# Autodesk Inventor assembly: Case
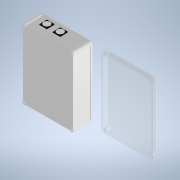
[picture p0: Inventor's stored thumbnail of the model, 180x180]
Saved by Autodesk Inventor 2020 (Build 240168000, 168)
## iProperties
Created: 2019-12-11
Part Number: Case
Document SubType Name: Assembly
Designer: nicoc
Author: nicoc
## Documents named in this file (12)
- D:\Repos\P5-AIonFPGA\cad\Case\Case.iam
- D:\Repos\P5-AIonFPGA\cad\Case\Ultra96\PWB_USDEV1-1_FINAL.iam
- D:\Repos\P5-AIonFPGA\cad\Case\Terminalblock\Terminalblock.iam
- D:\Repos\P5-AIonFPGA\cad\Case\SlottedWiring\SlottexWiring200mm.ipt
- D:\Repos\P5-AIonFPGA\cad\Case\SlottedWiring\SlottexWiring110mm.ipt
- D:\Repos\P5-AIonFPGA\cad\Case\Ventilator\Filter.ipt
- D:\Repos\P5-AIonFPGA\cad\Case\Fibox_PC_3828 _3_T_Bottom.ipt
- D:\Repos\P5-AIonFPGA\cad\Case\Fibox_PC_3828 _3_T_Top.ipt
- D:\Repos\P5-AIonFPGA\cad\Case\Ventilator\Fan_40x40x20.iam
- D:\Repos\P5-AIonFPGA\cad\Case\Ventilator\Filter40x40x20.ipt
- D:\Repos\P5-AIonFPGA\cad\Case\Ventilator\Fan_60x60x25.ipt
- D:\Repos\P5-AIonFPGA\cad\Case\Ultra96\USBCable.ipt
## Components (15 placed, 11 different names)
1. PWB_USDEV1-1_FINAL:1 [sub-assembly] — Mate:4, Mate:5, Mate:8, Mate:23, Flush:20, Flush:21
2. Terminalblock:1 [sub-assembly] — Mate:6, Mate:7
3. SlottexWiring200mm:1 — Mate:2, Flush:2, Flush:3, Flush:4
4. SlottexWiring200mm:2 — Mate:1, Flush:1, Flush:4, Mate:7, Mate:8
5. SlottexWiring110mm:1 — Mate:1, Flush:1, Mate:2, Flush:2, Flush:3, Mate:3, Mate:5
6. Filter:1 — Mate:15
7. Filter:2 — Mate:14, Mate:22, Flush:18, Flush:19
8. Fibox_PC_3828 _3_T_Bottom:1 — Mate:3, Mate:4, Mate:6, Mate:14, Mate:15, Mate:16, Mate:20, Mate:21
9. Fibox_PC_3828 _3_T_Top:1 — Mate:21
10. Fan_40x40x20:1 [sub-assembly] — Mate:17, Flush:11, Flush:12
11. Filter40x40x20:1 — Mate:16, Mate:17, Flush:11, Flush:12, Flush:17
12. Fan_40x40x20:3 [sub-assembly]
13. Filter40x40x20:3 — Mate:20, Flush:17
14. Fan_60x60x25:1 — Mate:22, Flush:18, Flush:19
15. USBCable:1 — Mate:23, Flush:20, Flush:21
## Relationships (30: Mate 17, Flush 13)
- Mate:1: SlottexWiring200mm:2 ↔ SlottexWiring110mm:1
- Flush:1: SlottexWiring200mm:2 ↔ SlottexWiring110mm:1
- Mate:2: SlottexWiring200mm:1 ↔ SlottexWiring110mm:1
- Flush:2: SlottexWiring200mm:1 ↔ SlottexWiring110mm:1
- Flush:3: SlottexWiring200mm:1 ↔ SlottexWiring110mm:1
- Flush:4: SlottexWiring200mm:1 ↔ SlottexWiring200mm:2
- Mate:3: SlottexWiring110mm:1 ↔ Fibox_PC_3828 _3_T_Bottom:1
- Mate:4: PWB_USDEV1-1_FINAL:1 ↔ Fibox_PC_3828 _3_T_Bottom:1
- Mate:5 (40 mm): PWB_USDEV1-1_FINAL:1 ↔ SlottexWiring110mm:1
- Mate:6: Terminalblock:1 ↔ Fibox_PC_3828 _3_T_Bottom:1
- Mate:7 (10 mm): Terminalblock:1 ↔ SlottexWiring200mm:2
- Mate:8 (12.5 mm): PWB_USDEV1-1_FINAL:1 ↔ SlottexWiring200mm:2
- Mate:14: Filter:2 ↔ Fibox_PC_3828 _3_T_Bottom:1
- Mate:15: Filter:1 ↔ Fibox_PC_3828 _3_T_Bottom:1
- Mate:16: Fibox_PC_3828 _3_T_Bottom:1 ↔ Filter40x40x20:1
- Mate:17 (7 mm): Fan_40x40x20:1 ↔ Filter40x40x20:1
- Flush:11: Fan_40x40x20:1 ↔ Filter40x40x20:1
- Flush:12: Fan_40x40x20:1 ↔ Filter40x40x20:1
- [Mate] (7 mm): Fan_40x40x20:3 ↔ Filter40x40x20:3
- [Flush]: Fan_40x40x20:3 ↔ Filter40x40x20:3
- [Flush]: Fan_40x40x20:3 ↔ Filter40x40x20:3
- Mate:20: Fibox_PC_3828 _3_T_Bottom:1 ↔ Filter40x40x20:3
- Flush:17: Filter40x40x20:1 ↔ Filter40x40x20:3
- Mate:21: Fibox_PC_3828 _3_T_Bottom:1 ↔ Fibox_PC_3828 _3_T_Top:1
- Mate:22 (7 mm): Filter:2 ↔ Fan_60x60x25:1
- Flush:18: Filter:2 ↔ Fan_60x60x25:1
- Flush:19: Filter:2 ↔ Fan_60x60x25:1
- Mate:23: PWB_USDEV1-1_FINAL:1 ↔ USBCable:1
- Flush:20: PWB_USDEV1-1_FINAL:1 ↔ USBCable:1
- Flush:21 (1 mm): PWB_USDEV1-1_FINAL:1 ↔ USBCable:1
## Named parameters: d109_d103 = 7 mm, d110_d104 = 0 mm, d111_d105 = 0 mm
